# Autodesk Inventor assembly: STI Hybrid 98 Cryocooler Assembly
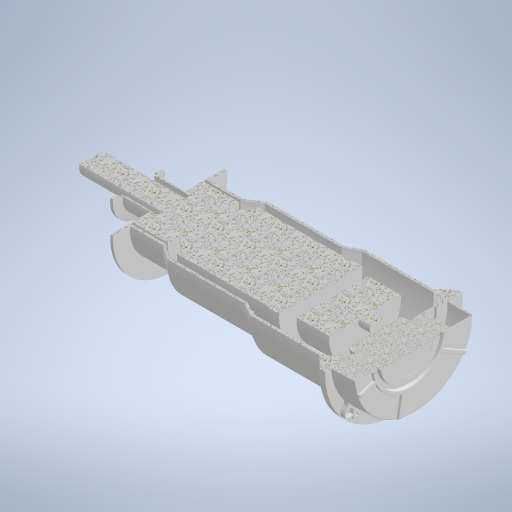
[picture p0: Inventor's stored thumbnail of the model, 512x512]
Saved by Autodesk Inventor 2023 (Build 270158000, 158)
## iProperties
Created: 2024-05-02
Part Number: STI Hybrid 98 Cryocooler Assembly
Document SubType Name: Assembly
Designer: incep
Author: incep
## Documents named in this file (4)
- C:\Users\incep\OneDrive\Desktop\3D Printer Stuff\STI Hybrid 98 Cryocooler Assembly.iam
- C:\Users\incep\OneDrive\Desktop\3D Printer Stuff\STI Hybrid 98 Cryocooler.ipt
- C:\Users\incep\OneDrive\Desktop\3D Printer Stuff\STI Hybrid 98 Cooling Shroud.ipt
- C:\Users\incep\OneDrive\Desktop\3D Printer Stuff\OAB800AN_m0.ipt
## Components (3 placed, 3 different names)
1. STI Hybrid 98 Cryocooler:1 — Flush:1, Flush:2, Flush:3, Mate:1, Mate:2, Mate:3, Mate:4, Mate:5, Flush:4, Flush:5
2. STI Hybrid 98 Cooling Shroud:1 — Mate:5, Flush:4, Flush:5, Mate:6, Mate:7
3. OAB800AN_m0:1 — Mate:6, Mate:7
## Relationships (12: Mate 7, Flush 5)
- Flush:1: STI Hybrid 98 Cryocooler:1
- Flush:2: STI Hybrid 98 Cryocooler:1
- Flush:3: STI Hybrid 98 Cryocooler:1
- Mate:1: STI Hybrid 98 Cryocooler:1
- Mate:2: STI Hybrid 98 Cryocooler:1
- Mate:3: STI Hybrid 98 Cryocooler:1
- Mate:4: STI Hybrid 98 Cryocooler:1
- Mate:5: STI Hybrid 98 Cryocooler:1 ↔ STI Hybrid 98 Cooling Shroud:1
- Flush:4: STI Hybrid 98 Cryocooler:1 ↔ STI Hybrid 98 Cooling Shroud:1
- Flush:5: STI Hybrid 98 Cryocooler:1 ↔ STI Hybrid 98 Cooling Shroud:1
- Mate:6: STI Hybrid 98 Cooling Shroud:1 ↔ OAB800AN_m0:1
- Mate:7: STI Hybrid 98 Cooling Shroud:1 ↔ OAB800AN_m0:1
